# Autodesk Inventor assembly: Lift Cart
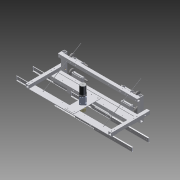
[picture p0: Inventor's stored thumbnail of the model, 180x180]
Saved by Autodesk Inventor 2015 (Build 190159000, 159)
## iProperties
Created: 2015-01-27
Part Number: Lift Cart
Document SubType Name: Assembly
Designer: Admin
Author: Admin
## Documents named in this file (16)
- C:\Users\Jarod\Documents\Robotics\FRC\2015\CAD\Robot\Lift Cart\Lift Cart.iam
- C:\Users\Jarod\Documents\Robotics\FRC\2015\CAD\Robot\Lift Cart\1x1 horizontal.ipt
- C:\Users\Jarod\Documents\Robotics\FRC\2015\CAD\Robot\Lift Cart\1x1 vertical.ipt
- C:\Users\Jarod\Documents\Robotics\FRC\2015\CAD\Robot\Lift Cart\1x1 lengthwise.ipt
- C:\Users\Jarod\Documents\Robotics\FRC\2015\CAD\Robot\Lift Cart\2x2 angle rail support.ipt
- C:\Users\Jarod\Documents\Robotics\FRC\2015\CAD\Robot\Lift Cart\motor support plate.ipt
- C:\Users\Jarod\Documents\Robotics\FRC\2015\CAD\Robot\Lift Cart\garage door 2in roller.ipt
- C:\Users\Jarod\Documents\Robotics\FRC\2015\CAD\Robot\Lift Cart\garage door hinge.ipt
- C:\Users\Jarod\Documents\Robotics\FRC\2015\CAD\Robot\Lift Cart\Imported Components\Versaplanetary Gearbox\Versaplanetary Gearbox.iam
- C:\Users\Jarod\Documents\Robotics\FRC\2015\CAD\Robot\Lift Cart\pinion.ipt
- C:\Users\Jarod\Documents\Robotics\FRC\2015\CAD\Robot\Lift Cart\Accuride Slider (301-12)\Accuride Slider (301-12).iam
- C:\Users\Jarod\Documents\Robotics\FRC\2015\CAD\Robot\Lift Cart\Imported Components\0.5 Hex Shaft Collar\0.5 Hex Shaft Collar.ipt
- C:\Users\Jarod\Documents\Robotics\FRC\2015\CAD\Robot\Lift Cart\1x1 horizontal lower.ipt
- C:\Users\Jarod\Documents\Robotics\FRC\2015\CAD\Robot\Lift Cart\bushing.ipt
- C:\Users\Jarod\Documents\Robotics\FRC\2015\CAD\Robot\Lift Cart\spacer.ipt
- C:\Users\Jarod\Documents\Robotics\FRC\2015\CAD\Robot\Lift Cart\cable.ipt
## Components (30 placed, 15 different names)
1. 1x1 horizontal:1 — Mate:1, Flush:1, Flush:2, Flush:3, Mate:19, Mate:21, Flush:31, Mate:56, Flush:32, Mate:59, Mate:94, Flush:43, Mate:101, Mate:109
2. 1x1 horizontal lower:1 — Flush:33, Mate:95, Flush:44, Mate:116, Mate:117, Mate:118, Mate:119, Mate:120, Mate:121
3. 1x1 vertical:1 — Mate:1, Flush:1, Flush:2, Mate:68, Mate:69, Mate:90, Mate:91
4. 1x1 vertical:2 — Flush:3, Flush:33, Mate:94, Flush:43, Mate:95, Flush:44, Mate:96, Mate:97
5. 1x1 lengthwise:1 — Mate:8, Mate:9, Flush:23, Flush:37, Flush:38, Mate:67, Mate:68, Mate:69, Flush:42
6. 1x1 lengthwise:2 — Flush:36, Flush:41, Flush:42
7. bushing:1 — Mate:90, Mate:91, Mate:92, Mate:93
8. bushing:2 — Mate:96, Mate:97, Mate:98, Mate:99
9. spacer:1 — Mate:92, Mate:93
10. spacer:2 — Mate:98, Mate:99
11. 2x2 angle rail support:1 — Mate:8, Mate:11, Flush:23, Mate:39, Mate:50, Mate:51, Flush:36, Flush:37, Mate:66, Mate:70, Flush:41, Mate:100, Mate:102, Mate:110, Mate:111, Mate:115, Mate:126
12. 2x2 angle rail support:2 — Mate:9, Mate:43, Mate:52, Mate:53, Flush:38, Mate:67, Mate:71, Mate:127
13. motor support plate:1 — Mate:11, Mate:17, Mate:28, Mate:29, Mate:62, Mate:66, Mate:115
14. garage door 2in roller:1 — Mate:57, Mate:58
15. garage door 2in roller:2 — Mate:122, Mate:125
16. garage door 2in roller:3 — Mate:60, Mate:61
17. garage door 2in roller:4 — Mate:123, Mate:124
18. garage door hinge:1 — Mate:19, Flush:31, Mate:56, Mate:57, Mate:58
19. garage door hinge:2 — Mate:116, Mate:117, Mate:118, Mate:122, Mate:125
20. garage door hinge:3 — Mate:21, Flush:32, Mate:59, Mate:60, Mate:61
21. garage door hinge:4 — Mate:119, Mate:120, Mate:121, Mate:123, Mate:124
22. Versaplanetary Gearbox:1 [sub-assembly] — Mate:17, Mate:18, Mate:28, Mate:29
23. pinion:1 — Mate:18, Mate:62, Mate:63, Mate:64
24. 0.5 Hex Shaft Collar:1 — Mate:63, Mate:64
25. Accuride Slider (301-12):1 [sub-assembly] — Mate:39, Flush:27, Flush:28, Mate:50, Mate:51, Mate:126
26. Accuride Slider (301-12):2 [sub-assembly] — Flush:27, Flush:28, Mate:70
27. Accuride Slider (301-12):3 [sub-assembly] — Flush:26, Flush:29, Mate:71
28. Accuride Slider (301-12):4 [sub-assembly] — Flush:26, Mate:43, Flush:29, Mate:52, Mate:53, Mate:127
29. cable:1 — Mate:100, Mate:101, Mate:102
30. cable:4 — Mate:109, Mate:110, Mate:111
## Relationships (78: Mate 60, Flush 18)
- Mate:1: 1x1 horizontal:1 ↔ 1x1 vertical:1
- Flush:1: 1x1 horizontal:1 ↔ 1x1 vertical:1
- Flush:2: 1x1 horizontal:1 ↔ 1x1 vertical:1
- Flush:3: 1x1 horizontal:1 ↔ 1x1 vertical:2
- Mate:8: 1x1 lengthwise:1 ↔ 2x2 angle rail support:1
- Mate:9: 1x1 lengthwise:1 ↔ 2x2 angle rail support:2
- Mate:11: 2x2 angle rail support:1 ↔ motor support plate:1
- Mate:17: motor support plate:1 ↔ Versaplanetary Gearbox:1
- Mate:18: Versaplanetary Gearbox:1 ↔ pinion:1
- Mate:19: 1x1 horizontal:1 ↔ garage door hinge:1
- Mate:21: 1x1 horizontal:1 ↔ garage door hinge:3
- Flush:23: 1x1 lengthwise:1 ↔ 2x2 angle rail support:1
- Mate:28: motor support plate:1 ↔ Versaplanetary Gearbox:1
- Mate:29: motor support plate:1 ↔ Versaplanetary Gearbox:1
- Flush:26: Accuride Slider (301-12):3 ↔ Accuride Slider (301-12):4
- Mate:39: 2x2 angle rail support:1 ↔ Accuride Slider (301-12):1
- Flush:27: Accuride Slider (301-12):1 ↔ Accuride Slider (301-12):2
- Flush:28: Accuride Slider (301-12):1 ↔ Accuride Slider (301-12):2
- Mate:43: 2x2 angle rail support:2 ↔ Accuride Slider (301-12):4
- Flush:29: Accuride Slider (301-12):3 ↔ Accuride Slider (301-12):4
- Mate:50 (34.925 mm): 2x2 angle rail support:1 ↔ Accuride Slider (301-12):1
- Mate:51 (34.925 mm): 2x2 angle rail support:1 ↔ Accuride Slider (301-12):1
- Mate:52 (34.925 mm): 2x2 angle rail support:2 ↔ Accuride Slider (301-12):4
- Mate:53 (34.925 mm): 2x2 angle rail support:2 ↔ Accuride Slider (301-12):4
- Flush:31 (-25.4 mm): 1x1 horizontal:1 ↔ garage door hinge:1
- Mate:56: 1x1 horizontal:1 ↔ garage door hinge:1
- Mate:57: garage door 2in roller:1 ↔ garage door hinge:1
- Mate:58 (3.175 mm): garage door 2in roller:1 ↔ garage door hinge:1
- Flush:32 (-25.4 mm): 1x1 horizontal:1 ↔ garage door hinge:3
- Mate:59: 1x1 horizontal:1 ↔ garage door hinge:3
- Mate:60: garage door 2in roller:3 ↔ garage door hinge:3
- Mate:61 (3.175 mm): garage door 2in roller:3 ↔ garage door hinge:3
- Mate:62 (9.525 mm): motor support plate:1 ↔ pinion:1
- Mate:63: pinion:1 ↔ 0.5 Hex Shaft Collar:1
- Mate:64: pinion:1 ↔ 0.5 Hex Shaft Collar:1
- Flush:33: 1x1 horizontal lower:1 ↔ 1x1 vertical:2
- Flush:36: 1x1 lengthwise:2 ↔ 2x2 angle rail support:1
- Flush:37: 1x1 lengthwise:1 ↔ 2x2 angle rail support:1
- Flush:38: 1x1 lengthwise:1 ↔ 2x2 angle rail support:2
- Mate:66: 2x2 angle rail support:1 ↔ motor support plate:1
- Mate:67: 1x1 lengthwise:1 ↔ 2x2 angle rail support:2
- Mate:68: 1x1 vertical:1 ↔ 1x1 lengthwise:1
- Mate:69: 1x1 vertical:1 ↔ 1x1 lengthwise:1
- Mate:70: 2x2 angle rail support:1 ↔ Accuride Slider (301-12):2
- Mate:71: 2x2 angle rail support:2 ↔ Accuride Slider (301-12):3
- Mate:90: 1x1 vertical:1 ↔ bushing:1
- Mate:91: 1x1 vertical:1 ↔ bushing:1
- Mate:92: bushing:1 ↔ spacer:1
- Mate:93: bushing:1 ↔ spacer:1
- Flush:41: 1x1 lengthwise:2 ↔ 2x2 angle rail support:1
- Flush:42: 1x1 lengthwise:1 ↔ 1x1 lengthwise:2
- Mate:94: 1x1 horizontal:1 ↔ 1x1 vertical:2
- Flush:43: 1x1 horizontal:1 ↔ 1x1 vertical:2
- Mate:95: 1x1 horizontal lower:1 ↔ 1x1 vertical:2
- Flush:44 (25.4 mm): 1x1 horizontal lower:1 ↔ 1x1 vertical:2
- Mate:96: 1x1 vertical:2 ↔ bushing:2
- Mate:97: 1x1 vertical:2 ↔ bushing:2
- Mate:98: bushing:2 ↔ spacer:2
- Mate:99: bushing:2 ↔ spacer:2
- Mate:100: 2x2 angle rail support:1 ↔ cable:1
- Mate:101: 1x1 horizontal:1 ↔ cable:1
- Mate:102: 2x2 angle rail support:1 ↔ cable:1
- Mate:109: 1x1 horizontal:1 ↔ cable:4
- Mate:110: 2x2 angle rail support:1 ↔ cable:4
- Mate:111: 2x2 angle rail support:1 ↔ cable:4
- Mate:115: 2x2 angle rail support:1 ↔ motor support plate:1
- Mate:116: 1x1 horizontal lower:1 ↔ garage door hinge:2
- Mate:117: 1x1 horizontal lower:1 ↔ garage door hinge:2
- Mate:118: 1x1 horizontal lower:1 ↔ garage door hinge:2
- Mate:119: 1x1 horizontal lower:1 ↔ garage door hinge:4
- Mate:120: 1x1 horizontal lower:1 ↔ garage door hinge:4
- Mate:121: 1x1 horizontal lower:1 ↔ garage door hinge:4
- Mate:122: garage door 2in roller:2 ↔ garage door hinge:2
- Mate:123: garage door 2in roller:4 ↔ garage door hinge:4
- Mate:124 (3.175 mm): garage door 2in roller:4 ↔ garage door hinge:4
- Mate:125 (3.175 mm): garage door 2in roller:2 ↔ garage door hinge:2
- Mate:126: 2x2 angle rail support:1 ↔ Accuride Slider (301-12):1
- Mate:127: 2x2 angle rail support:2 ↔ Accuride Slider (301-12):4
